# Autodesk Inventor assembly: Zlozenie_prowadnica_na_tlok_nakretka
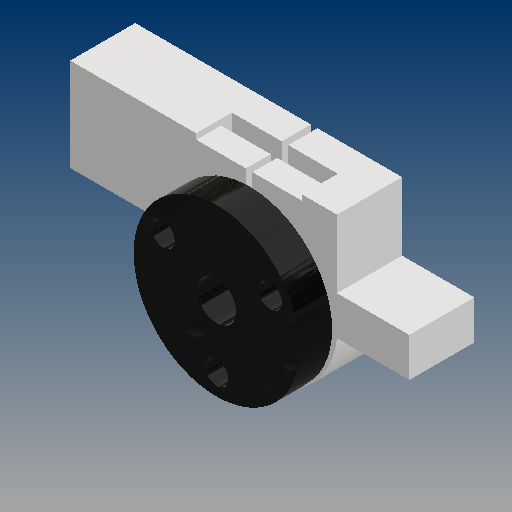
[picture p0: Inventor's stored thumbnail of the model, 512x512]
Saved by Autodesk Inventor 2021 (Build 250183000, 183)
## iProperties
Created: 2022-10-06
Part Number: Zlozenie_prowadnica_na_tlok_nakretka
Document SubType Name: Assembly
Designer: agnpi
Author: agnpi
## Documents named in this file (3)
- E:\Users\agnpi\Desktop\lekcje\SEMESTR VII\Inventor inzynierka\Zlozenie_prowadnica_na_tlok_nakretka.iam
- E:\Users\agnpi\Desktop\lekcje\SEMESTR VII\Inventor inzynierka\Prowadnica_tloka.ipt
- E:\Users\agnpi\Desktop\lekcje\SEMESTR VII\Inventor inzynierka\Nakretka_prowadnica_tloka.ipt
## Components (2 placed, 2 different names)
1. Prowadnica_tloka:1 — Mate:1, Mate:2, Mate:3
2. Nakretka_prowadnica_tloka:1 — Mate:1, Mate:2, Mate:3
## Relationships (3: Mate 3)
- Mate:1: Prowadnica_tloka:1 ↔ Nakretka_prowadnica_tloka:1
- Mate:2: Prowadnica_tloka:1 ↔ Nakretka_prowadnica_tloka:1
- Mate:3: Prowadnica_tloka:1 ↔ Nakretka_prowadnica_tloka:1
